# Autodesk Inventor assembly: 40-J4
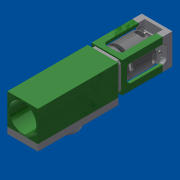
[picture p0: Inventor's stored thumbnail of the model, 180x180]
Saved by Autodesk Inventor 2018 (Build 220112000, 112)
## iProperties
Created: 2020-06-07
Part Number: 40-J4
Document SubType Name: Assembly
Designer: Bunny320
Author: Bunny320
## Documents named in this file (4)
- C:\Users\Bunny320\Desktop\sechs\4-CAD\40-J4.iam
- C:\Users\Bunny320\Desktop\sechs\4-CAD\motor unit 2820.iam
- C:\Users\Bunny320\Desktop\sechs\4-CAD\401-flange.ipt
- C:\Users\Bunny320\Desktop\sechs\4-CAD\402-gearbox-housing.ipt
## Components (3 placed, 3 different names)
1. motor unit 2820:1 [sub-assembly] — Flush:1, Flush:2, Flush:3, Mate:1, Mate:2, Mate:3, Mate:4
2. 401-flange:1 — Mate:1, Flush:5, Flush:6
3. 402-gearbox-housing:1 — Mate:2, Mate:3, Mate:4, Flush:5, Flush:6
## Relationships (9: Flush 5, Mate 4)
- Flush:1: motor unit 2820:1
- Flush:2: motor unit 2820:1
- Flush:3: motor unit 2820:1
- Mate:1: motor unit 2820:1 ↔ 401-flange:1
- Mate:2: motor unit 2820:1 ↔ 402-gearbox-housing:1
- Mate:3: motor unit 2820:1 ↔ 402-gearbox-housing:1
- Mate:4: motor unit 2820:1 ↔ 402-gearbox-housing:1
- Flush:5: 401-flange:1 ↔ 402-gearbox-housing:1
- Flush:6: 401-flange:1 ↔ 402-gearbox-housing:1
